# Autodesk Inventor assembly: ENSAMBLE FINAL JIMENA OSOY
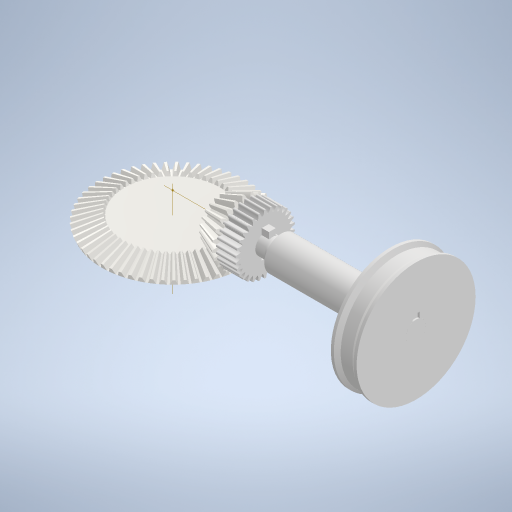
[picture p0: Inventor's stored thumbnail of the model, 512x512]
Saved by Autodesk Inventor 2024 (Build 280153000, 153)
## iProperties
Created: 2024-03-19
Part Number: ENSAMBLE FINAL JIMENA OSOY
Document SubType Name: Assembly
Designer: Jime
Author: Jime
## Documents named in this file (6)
- C:\Users\50255\Desktop\UNIVERSIDAD\QUINTO SEMESTRE\DINÁMICA\LAB\ENSAMBLE FINAL JIMENA OSOY.iam
- C:\Users\50255\Downloads\ENGRANE.ipt
- C:\Users\50255\Downloads\CUÑA.ipt
- C:\Users\50255\Downloads\EJE_CUÑEROS.ipt
- C:\Users\50255\Downloads\POLEA.ipt
- C:\Users\50255\Desktop\UNIVERSIDAD\QUINTO SEMESTRE\DINÁMICA\LAB\ENSAMBLE FINAL JIMENA OSOY\Design Accelerator\Bevel Gears1.iam
## Components (6 placed, 5 different names)
1. EJE_CUÑEROS:2 — Cylindrical:3, Flush:5, Rigid:4, Rigid:5, Cylindrical:4, Mate:1, Mate:2, Flush:6, Rotational:1
2. CUÑA:4 — Rigid:4
3. CUÑA:5 — Rigid:5
4. ENGRANE:2 — Cylindrical:3, Flush:5
5. POLEA:1 — Cylindrical:4, Mate:1, Mate:2, Flush:6
6. Bevel Gears:1 [sub-assembly] — Rotational:1
## Relationships (9: CylindricalJoint 2, Flush 2, WeldJoint 2, Mate 2, RevoluteJoint 1)
- Cylindrical:3: EJE_CUÑEROS:2 ↔ ENGRANE:2
- Flush:5: EJE_CUÑEROS:2 ↔ ENGRANE:2
- Rigid:4 [WeldJoint]: EJE_CUÑEROS:2 ↔ CUÑA:4
- Rigid:5 [WeldJoint]: EJE_CUÑEROS:2 ↔ CUÑA:5
- Cylindrical:4: EJE_CUÑEROS:2 ↔ POLEA:1
- Mate:1: EJE_CUÑEROS:2 ↔ POLEA:1
- Mate:2: EJE_CUÑEROS:2 ↔ POLEA:1
- Flush:6: EJE_CUÑEROS:2 ↔ POLEA:1
- Rotational:1 [RevoluteJoint]: EJE_CUÑEROS:2 ↔ Bevel Gears:1
